# Autodesk Inventor assembly: ASY PNS-722 charging hatch
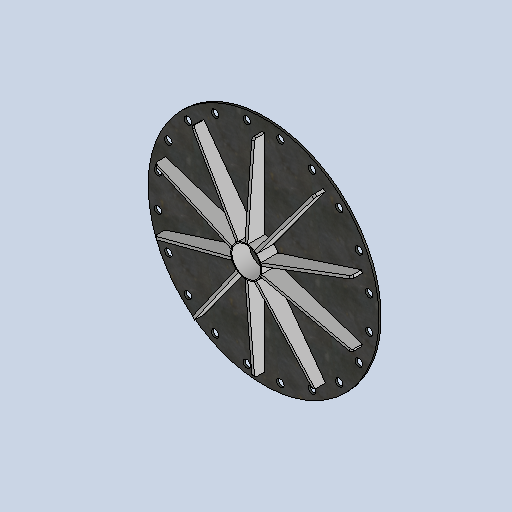
[picture p0: Inventor's stored thumbnail of the model, 512x512]
Saved by Autodesk Inventor 2025.1 (Build 291241020, 241B)
## iProperties
Created: 2025-04-22
Part Number: ASY PNS-722 charging hatch
Document SubType Name: Assembly
Designer: user
Author: user
## Documents named in this file (4)
- C:\Users\user\YandexDisk-badmisterfox\home pc\Inventor\PNS2-Panaevsk\Filter D1000\ASY PNS-722 charging hatch.iam
- C:\Users\user\YandexDisk-badmisterfox\home pc\Inventor\PNS2-Panaevsk\Filter D1200\PNS-721 charging hatch D1200.ipt
- C:\Users\user\YandexDisk-badmisterfox\home pc\Inventor\PNS2-Panaevsk\Filter D1200\PNS-725 charging hatch reinf D1200.ipt
- C:\Users\user\YandexDisk-badmisterfox\home pc\Inventor\PNS2-Panaevsk\Filter D1200\PNS- 727 hatch tube .ipt
## Components (12 placed, 3 different names)
1. PNS-721 charging hatch D1200.ipt:1 — Rigid:1, Flush:1
2. PNS- 727 hatch tube :1 — Rigid:1
3. PNS-725 charging hatch reinf D1200:1 — Mate:1, Flush:1, Mate:2, Mate:3
4. PNS-725 charging hatch reinf D1200:2
5. PNS-725 charging hatch reinf D1200:3
6. PNS-725 charging hatch reinf D1200:4
7. PNS-725 charging hatch reinf D1200:5
8. PNS-725 charging hatch reinf D1200:6
9. PNS-725 charging hatch reinf D1200:7
10. PNS-725 charging hatch reinf D1200:8
11. PNS-725 charging hatch reinf D1200:9
12. PNS-725 charging hatch reinf D1200:10
## Component patterns: (10 elements, first: PNS-725 charging hatch reinf D1200:1)
## Relationships (5: Mate 3, WeldJoint 1, Flush 1)
- Rigid:1 [WeldJoint]: PNS-721 charging hatch D1200.ipt:1 ↔ PNS- 727 hatch tube :1
- Mate:1: PNS-725 charging hatch reinf D1200:1
- Flush:1: PNS-721 charging hatch D1200.ipt:1 ↔ PNS-725 charging hatch reinf D1200:1
- Mate:2: PNS-725 charging hatch reinf D1200:1
- Mate:3: PNS-725 charging hatch reinf D1200:1
